# Autodesk Inventor assembly: DynamixelXM540_no_idler_drivable
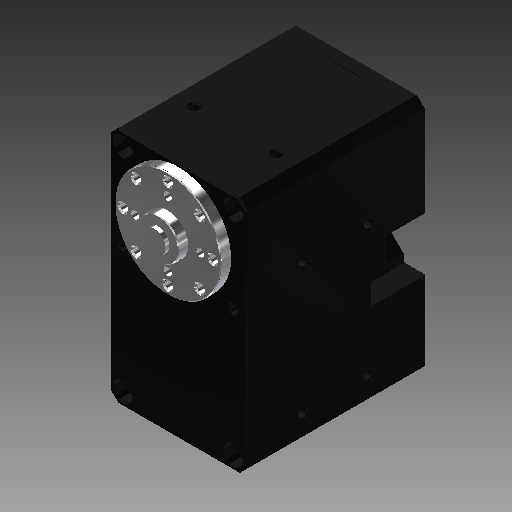
[picture p0: Inventor's stored thumbnail of the model, 512x512]
Saved by Autodesk Inventor 2023 (Build 270158000, 158)
## iProperties
Created: 2018-06-30
Part Number: DynamixelXM540_no_idler_drivable
Material: 一般
Document SubType Name: Assembly
Designer: TAKEMORI
Mass: 158.355 g
Surface Area: 205.744 cm^2
Volume: 58.65 cm^3
Density: 2.7 g/cm^3
Author: TAKEMORI
## Documents named in this file (3)
- C:\Users\michi\OneDrive - Kyoto University\lab\6_SHINOBI\FUHGA3\Design_Mechanism\Dynamixel\X540\DynamixelXM540_no_idler_drivable.iam
- C:\Users\michi\OneDrive - Kyoto University\lab\6_SHINOBI\FUHGA3\Design_Mechanism\Dynamixel\X540\DynamixelXM540_without_hone.ipt
- C:\Users\michi\OneDrive - Kyoto University\lab\6_SHINOBI\FUHGA3\Design_Mechanism\Dynamixel\X540\DynamixelXM540_hone.ipt
## Components (2 placed, 2 different names)
1. DynamixelXM540_without_hone:1 — フラッシュ:1, フラッシュ:2, フラッシュ:3, 挿入:1
2. DynamixelXM540_hone:1 — 挿入:1
## Relationships (4: Flush 3, Insert 1)
- フラッシュ:1 [Flush]: DynamixelXM540_without_hone:1
- フラッシュ:2 [Flush]: DynamixelXM540_without_hone:1
- フラッシュ:3 [Flush]: DynamixelXM540_without_hone:1
- 挿入:1 [Insert]: DynamixelXM540_without_hone:1 ↔ DynamixelXM540_hone:1
